# Autodesk Inventor assembly: CaseAssembly
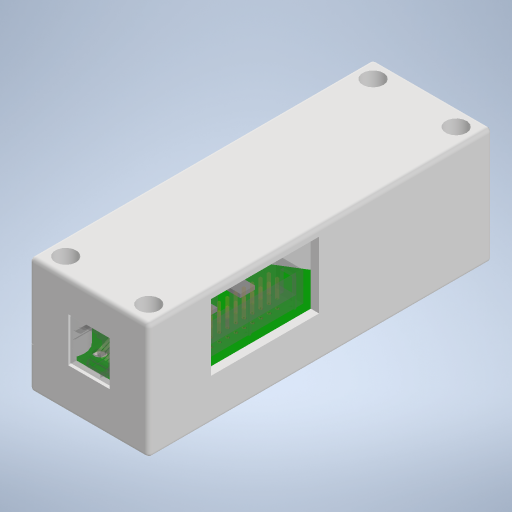
[picture p0: Inventor's stored thumbnail of the model, 512x512]
Saved by Autodesk Inventor 2023 (Build 270158000, 158)
## iProperties
Created: 2022-10-24
Part Number: CaseAssembly
Document SubType Name: Assembly
Designer: Intern
Author: Intern
## Documents named in this file (4)
- C:\Users\Intern\Documents\GitHub\dtb-218\CaseAssembly.iam
- C:\Users\Intern\Documents\GitHub\dtb-218\CaseTop.ipt
- C:\Users\Intern\Documents\GitHub\dtb-218\dtb-218-AW1.ipt
- C:\Users\Intern\Documents\GitHub\dtb-218\CaseBottom.ipt
## Components (3 placed, 3 different names)
1. CaseTop:1 — Mate:1, Mate:2, Flush:1, Flush:2, Mate:3
2. dtb-218-AW1:1 — Mate:1, Mate:2
3. CaseBottom:1 — Flush:1, Flush:2, Mate:3
## Relationships (5: Mate 3, Flush 2)
- Mate:1: CaseTop:1 ↔ dtb-218-AW1:1
- Mate:2: CaseTop:1 ↔ dtb-218-AW1:1
- Flush:1: CaseTop:1 ↔ CaseBottom:1
- Flush:2: CaseTop:1 ↔ CaseBottom:1
- Mate:3: CaseTop:1 ↔ CaseBottom:1
